# Autodesk Inventor assembly: SSE2B-MX13-970
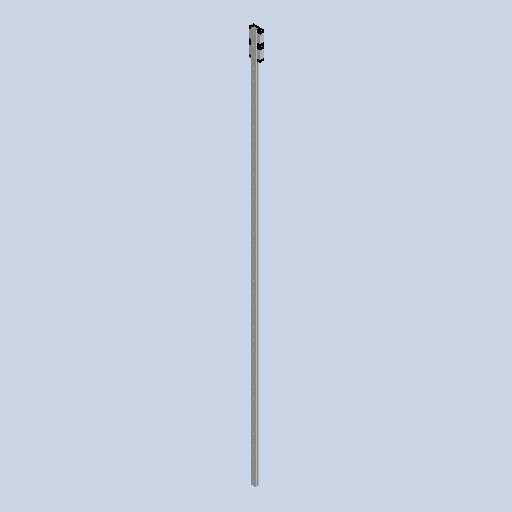
[picture p0: Inventor's stored thumbnail of the model, 512x512]
Saved by Autodesk Inventor 2025.2 (Build 292293000, 293)
## iProperties
Category: PARTsolutions
Company: MISUMI
Created: 2025-02-22
Part Number: SSE2B-MX13-970
Catalog Web Link: www.cadenas.de
Description: SSEB, SSEB-MX, SSE2B, SSE2B-MX, RSEB, RSE2B-Miniature Linear Guides Standard Blocks/Light Preload High Grade-L Selectable Type
Vendor: MISUMI
Document SubType Name: Assembly
Designer: psAdmin
Manufacturer: MISUMI
Mass: 89.2621 g
Surface Area: 540.949 cm^2
Volume: 89.2621 cm^3
Density: 1 g/cm^3
PSOL_IDENT_0: {$CADENAS_DATA/23d-libs/misumi/metric/06_linear_guides/re2b_asmtab.prj},265 {VTYP=3D},{STYP=ASSTAB},
PSOL_IDENT_1: {NB=SSE2B-MX13-970},{LINA=SSE2B-MX13-970},{NN=SSEB, SSEB-MX, SSE2B, SSE2B-MX, RSEB, RSE2B},{DATE=04.
PSOL_IDENT_2: 04.2024 07:12:35},{GEOMDATE=07.03.2024 00:33:43},{VERSION=},{LINEID=230},{WBVAR=ST,MAT,MX,NOB,GREASE
PSOL_IDENT_3: ,LS,ALT1,ALT2,ALT3,ALT4},{WBNUMERIC=LS}  {NB=SSE2B-MX13-970},{LINA=SSE2B-MX13-970},{KT=DUMMY},{PN=SS
PSOL_IDENT_4: E2B-MX13-970},{RT=B},{TYPE=SSE2B},{ST=S},{MAT=S},{MX=-MX},{MXALG='', 'w/o MX(Lubrication unit)', '-M
PSOL_IDENT_5: X', 'with MX(Lubrication unit)'},{NOB=2},{H=13},{GREASE=},{GREASEALG='','Normal'},{LT=Selectable},{L
PSOL_IDENT_6: S=970},{HARD=56HRC~},{W=27},{L1=33.9},{B=20},{C=15},{SLL=M3x3.5},{L2=19.9},{K=10.0},{CBB=0.5},{W1=12
PSOL_IDENT_7: },{W2=7.5},{H1=7.5},{CAA=0.5},{DD1DD2HH=3.5x6x4.5},{F=25},{G=10.0},{ALT1=},{ALT1ALG= '', 'w/o MC (Ta
PSOL_IDENT_8: pped Holes)' },{MC=M4},{ALT2=},{ALT2L=5.0},{ALT2N=5},{M=39},{LL=},{L0=95,120,145,170,195,220,245,270
PSOL_IDENT_9: ,295,320,345,370,395,420,445,470,495,520,545,570,595,620,645,670,695,720,745,770,795,820,845,870,895
PSOL_IDENT_10: ,920,945,970},{REC1=   '','w/o Rail Ends Cut alteration','-LLC','with LLC (Left End Cut)','-RLC','wi
PSOL_IDENT_11: th RLC (Right End Cut)','-LLC-RLC','with Both End Cut'   },{ST1='S', 'w/o Surface Treatment','R','Lo
PSOL_IDENT_12: w Temperature Black Chrome Plating'},{MAT2='S','Stainless Steel'},{ALT3=},{ALT3ALG= '' , 'w/o WC (Pa
PSOL_IDENT_13: ir of Rails)' , '-WC' , 'with WC (Set Pair of Rails)' },{ALT4=},{ALT4ALG= '','N/A' },{PPATH=seb_seri
PSOL_IDENT_14: es/seb_asmtpl.prj}
NB: SSE2B-MX13-970
NN: SSEB, SSEB-MX, SSE2B, SSE2B-MX, RSEB, RSE2B
NT: Miniature Linear Guides Standard Blocks/Light Preload High Grade-L Selectable Type
NBSYN: $PN.
LINA: SSE2B-MX13-970
CATALOG: Misumi
PN: SSE2B-MX13-970
ST: w/o Surface Treatment
MAT: Stainless Steel
MX: with MX(Lubrication unit)
NOB: 2
H: 13
GREASE: Normal
LS: 970
W: 27
L1: 33.9
B: 20
C: 15
SLL: M3x3.5
L2: 19.9
K: 10
CBB: 0.5
W1: 12
W2: 7.5
H1: 7.5
CAA: 0.5
DD1DD2HH: 3.5x6x4.5
F: 25
G: 10
ALT1: w/o MC (Tapped Holes)
ALT2: w/o Rail Ends Cut alteration
ALT3: w/o WC (Pair of Rails)
ALT4: N/A
SUPPLIER: MISUMI
ARTICLENO: SSE2B-MX13-970
BOMINFO: SSE2B-MX13-970
CREATOR: CADENAS GmbH
Title: SSE2B-MX13-970
Author: Cadenas PARTsolutions
Comments: Miniature Linear Guides Standard Blocks/Light Preload High Grade-L Selectable Type
## Documents named in this file (3)
- C:\Users\haruy\Documents\ロボコン\NHK2025\cad\nagahisa\belt_liner\SSE2B-MX13-970.iam
- C:\Users\haruy\Documents\ロボコン\NHK2025\cad\nagahisa\belt_liner\SSE2B-MX13-970_r.ipt
- C:\Users\haruy\Documents\ロボコン\NHK2025\cad\nagahisa\belt_liner\SSEB-MX13_b.ipt
## Components (3 placed, 2 different names)
1. SSE2B-MX13-970_r:1 — to_block_Z@1 <-> to_rail_Z@2, to_block_YZ@1 <-> to_rail_YZ@2, to_block_2_Z@1 <-> to_rail_Z@3, to_block_2_YZ@1 <-> to_rail_YZ@3
2. SSEB-MX13_b:1 — to_block_Z@1 <-> to_rail_Z@2, to_block_YZ@1 <-> to_rail_YZ@2, メイト:3
3. SSEB-MX13_b:2 — to_block_2_Z@1 <-> to_rail_Z@3, to_block_2_YZ@1 <-> to_rail_YZ@3, メイト:3
## Relationships (5: Mate 3, Angle 2)
- to_block_Z@1 <-> to_rail_Z@2 [Mate]: SSE2B-MX13-970_r:1 ↔ SSEB-MX13_b:1
- to_block_YZ@1 <-> to_rail_YZ@2 [Angle] (0 deg): SSE2B-MX13-970_r:1 ↔ SSEB-MX13_b:1
- to_block_2_Z@1 <-> to_rail_Z@3 [Mate]: SSE2B-MX13-970_r:1 ↔ SSEB-MX13_b:2
- to_block_2_YZ@1 <-> to_rail_YZ@3 [Angle] (0 deg): SSE2B-MX13-970_r:1 ↔ SSEB-MX13_b:2
- メイト:3 [Mate]: SSEB-MX13_b:1 ↔ SSEB-MX13_b:2
